# Autodesk Inventor assembly: [Top] Orbiter <1>
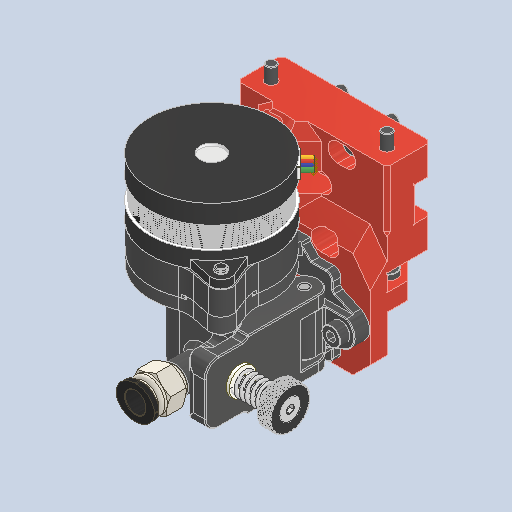
[picture p0: Inventor's stored thumbnail of the model, 512x512]
Saved by Autodesk Inventor 2022 (Build 260153000, 153)
## iProperties
Created: 2021-10-06
Part Number: [Top] Orbiter <1>
Document SubType Name: Assembly
Designer: Administrator
Title: [Top] Orbiter <1>
Author: Administrator
## Documents named in this file (6)
- Y:\Projects\Bibble0\Modified EVA Carriage\[Top] Orbiter _1_.iam
- Y:\Projects\Bibble0\Modified EVA Carriage\top_orbiter_mgn12.ipt
- Y:\Projects\Bibble0\Hardware\M3 x 35 mm.ipt
- Y:\Projects\Bibble0\Hardware\M3 x 10 mm.ipt
- Y:\Projects\Bibble0\Hardware\M3 Hex Nut.ipt
- Y:\Projects\Bibble0\Modified EVA Carriage\Orbiter Extruder V1.5.ipt
## Components (14 placed, 5 different names)
1. top_orbiter_mgn12:1 — Insert:1
2. RobertL-LDO-Vivedino-Orbiter-Extruder-V1.5 v36 <1>:1 — Insert:1, Mate:1
3. DIN 912 M3 35 mm:3
4. DIN 912 M3 10 mm:3 — Mate:1
5. M3  Hex nut :22
6. DIN 912 M3 10 mm:4
7. DIN 912 M3 10 mm:5
8. DIN 912 M3 10 mm:6
9. M3  Hex nut :23
10. DIN 912 M3 10 mm:7
11. DIN 912 M3 10 mm:8
12. DIN 912 M3 10 mm:9
13. DIN 912 M3 35 mm:4
14. DIN 912 M3 10 mm:10
## Relationships (2: Insert 1, Mate 1)
- Insert:1: top_orbiter_mgn12:1 ↔ RobertL-LDO-Vivedino-Orbiter-Extruder-V1.5 v36 <1>:1
- Mate:1: RobertL-LDO-Vivedino-Orbiter-Extruder-V1.5 v36 <1>:1 ↔ DIN 912 M3 10 mm:3
